# Autodesk Inventor assembly: 基本構造
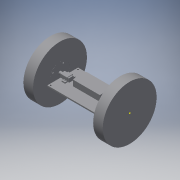
[picture p0: Inventor's stored thumbnail of the model, 180x180]
Saved by Autodesk Inventor 2017 (Build 210142000, 142)
## iProperties
Part Number: 基本構造
Material: 一般
Document SubType Name: Assembly
Designer: HISAAKI
Author: HISAAKI
## Documents named in this file (7)
- C:\Users\HISAAKI\Documents\LYNCS\CanSat\2017種子島\cansat-structure\基本構造.iam
- C:\Users\HISAAKI\Documents\LYNCS\CanSat\2017種子島\cansat-structure\基本板.ipt
- C:\Users\HISAAKI\Documents\LYNCS\CanSat\2017種子島\cansat-structure\既成部品\ブラケット.ipt
- C:\Users\HISAAKI\Documents\LYNCS\CanSat\2017種子島\cansat-structure\既成部品\モータ.ipt
- C:\Users\HISAAKI\Documents\LYNCS\CanSat\2017種子島\cansat-structure\ハブver1.1.ipt
- C:\Users\HISAAKI\Documents\LYNCS\CanSat\2017種子島\cansat-structure\タイヤスポンジ部分.ipt
- C:\Users\HISAAKI\Documents\LYNCS\CanSat\2017種子島\cansat-structure\既成部品\リポ電池.ipt
## Components (10 placed, 6 different names)
1. 基本板:1 — メイト:1, メイト:2, メイト:3, メイト:4, メイト:5, メイト:6, フラッシュ:1, フラッシュ:2, メイト:19
2. ブラケット:1 — メイト:1, メイト:2, メイト:6, メイト:9, メイト:10
3. ブラケット:2 — メイト:3, メイト:4, メイト:5, メイト:7, メイト:8
4. モータ:1 — フラッシュ:2, メイト:9, メイト:10, メイト:13, メイト:14
5. モータ:2 — フラッシュ:1, メイト:7, メイト:8, メイト:11, メイト:12
6. ハブver1.1:1 — メイト:11, メイト:12, メイト:17, メイト:18
7. ハブver1.1:2 — メイト:13, メイト:14, メイト:15, メイト:16
8. タイヤスポンジ部分:1 — メイト:15, メイト:16
9. タイヤスポンジ部分:2 — メイト:17, メイト:18
10. リポ電池:1 — メイト:19
## Relationships (21: Mate 19, Flush 2)
- メイト:1 [Mate]: 基本板:1 ↔ ブラケット:1
- メイト:2 [Mate]: 基本板:1 ↔ ブラケット:1
- メイト:3 [Mate]: 基本板:1 ↔ ブラケット:2
- メイト:4 [Mate]: 基本板:1 ↔ ブラケット:2
- メイト:5 [Mate]: 基本板:1 ↔ ブラケット:2
- メイト:6 [Mate]: 基本板:1 ↔ ブラケット:1
- フラッシュ:1 [Flush]: 基本板:1 ↔ モータ:2
- メイト:7 [Mate]: ブラケット:2 ↔ モータ:2
- メイト:8 [Mate]: ブラケット:2 ↔ モータ:2
- フラッシュ:2 [Flush]: 基本板:1 ↔ モータ:1
- メイト:9 [Mate]: ブラケット:1 ↔ モータ:1
- メイト:10 [Mate]: ブラケット:1 ↔ モータ:1
- メイト:11 [Mate]: モータ:2 ↔ ハブver1.1:1
- メイト:12 [Mate]: モータ:2 ↔ ハブver1.1:1
- メイト:13 [Mate]: モータ:1 ↔ ハブver1.1:2
- メイト:14 [Mate]: モータ:1 ↔ ハブver1.1:2
- メイト:15 [Mate]: ハブver1.1:2 ↔ タイヤスポンジ部分:1
- メイト:16 [Mate]: ハブver1.1:2 ↔ タイヤスポンジ部分:1
- メイト:17 [Mate]: ハブver1.1:1 ↔ タイヤスポンジ部分:2
- メイト:18 [Mate]: ハブver1.1:1 ↔ タイヤスポンジ部分:2
- メイト:19 [Mate]: 基本板:1 ↔ リポ電池:1
